# Autodesk Inventor assembly: Stopa v1
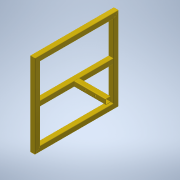
[picture p0: Inventor's stored thumbnail of the model, 180x180]
Saved by Autodesk Inventor 2021 (Build 250183000, 183)
## iProperties
Created: 2024-04-18
Part Number: Stopa v1
Document SubType Name: Assembly
Designer: Michal
Author: Michal
## Documents named in this file (4)
- C:\Users\Michal\Documents\GitHub\PNW_PhotoBoothFrame_3D\Stopa v1.iam
- C:\Users\Michal\Documents\GitHub\PNW_PhotoBoothFrame_3D\narrow high rectangular\beam 25x25x2 1-1.ipt
- C:\Users\Michal\Documents\GitHub\PNW_PhotoBoothFrame_3D\Stopa v1 profil 1.ipt
- C:\Users\Michal\Documents\GitHub\PNW_PhotoBoothFrame_3D\Stopa v1 profil 2.ipt
## Components (6 placed, 3 different names)
1. Stopa v1 profil 1:1 — Mate:1, Flush:1, Mate:2, Mate:5, Mate:6, Mate:8, Mate:10
2. Stopa v1 profil 1:2 — Mate:1, Flush:1, Mate:2, Flush:2, Mate:3, Mate:7, Flush:4
3. Stopa v1 profil 1:3 — Flush:2, Flush:3, Mate:3, Mate:4
4. Stopa v1 profil 1:4 — Flush:3, Mate:4, Mate:5, Mate:6, Mate:9
5. Stopa v1 profil 2:1 — Mate:7, Flush:4, Mate:11, Mate:12
6. beam 25x25x2 1-1:1 — Mate:12, Mate:13, Flush:5
## Relationships (18: Mate 13, Flush 5)
- Mate:1: Stopa v1 profil 1:1 ↔ Stopa v1 profil 1:2
- Flush:1: Stopa v1 profil 1:1 ↔ Stopa v1 profil 1:2
- Mate:2: Stopa v1 profil 1:1 ↔ Stopa v1 profil 1:2
- Flush:2: Stopa v1 profil 1:2 ↔ Stopa v1 profil 1:3
- Flush:3: Stopa v1 profil 1:3 ↔ Stopa v1 profil 1:4
- Mate:3: Stopa v1 profil 1:2 ↔ Stopa v1 profil 1:3
- Mate:4: Stopa v1 profil 1:3 ↔ Stopa v1 profil 1:4
- Mate:5: Stopa v1 profil 1:1 ↔ Stopa v1 profil 1:4
- Mate:6: Stopa v1 profil 1:1 ↔ Stopa v1 profil 1:4
- Mate:7: Stopa v1 profil 1:2 ↔ Stopa v1 profil 2:1
- Flush:4: Stopa v1 profil 1:2 ↔ Stopa v1 profil 2:1
- Mate:8: Stopa v1 profil 1:1
- Mate:9: Stopa v1 profil 1:4
- Mate:10: Stopa v1 profil 1:1
- Mate:11: Stopa v1 profil 2:1
- Mate:12: Stopa v1 profil 2:1 ↔ beam 25x25x2 1-1:1
- Mate:13: beam 25x25x2 1-1:1
- Flush:5: beam 25x25x2 1-1:1
